# Autodesk Inventor assembly: SPE1V1 Estructura
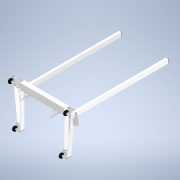
[picture p0: Inventor's stored thumbnail of the model, 180x180]
Saved by Autodesk Inventor 2021.2 (Build 252289000, 289)
## iProperties
Created: 2026-06-02
Part Number: SPE1V1 Estructura
Document SubType Name: Assembly
Designer: nelso
Author: nelso
## Documents named in this file (15)
- C:\Users\nelso\Desktop\Soporte-Paciente-Espinografia\Workspace\SPE1V1 Estructura.iam
- C:\Users\nelso\Desktop\Soporte-Paciente-Espinografia\Workspace\SP22V1 Tubo 40x80x1825mm.ipt
- C:\Users\nelso\Desktop\Soporte-Paciente-Espinografia\Workspace\SP21V1 Tubo 40x80x100mm.ipt
- C:\Users\nelso\Desktop\Soporte-Paciente-Espinografia\Workspace\SPE4V1 Rueda.iam
- C:\Users\nelso\Desktop\Soporte-Paciente-Espinografia\Workspace\SP23V1 Cobertora Derecha.ipt
- C:\Users\nelso\Desktop\Soporte-Paciente-Espinografia\Workspace\SP24V1 Cobertora Izquierda.ipt
- C:\Users\nelso\Desktop\Soporte-Paciente-Espinografia\Workspace\SP20V1 Tubo 80x120x790mm.ipt
- C:\Users\nelso\Desktop\Soporte-Paciente-Espinografia\Workspace\SP19V1 Tapacanto Delantero.ipt
- C:\Users\nelso\Desktop\Soporte-Paciente-Espinografia\Workspace\SP18V1 Tapacanto Superior.ipt
- C:\Users\nelso\Desktop\Soporte-Paciente-Espinografia\Workspace\RFPLUS8PO300.ipt
- C:\Users\nelso\Desktop\Soporte-Paciente-Espinografia\Workspace\SP17V1 Varilla Pedal.ipt
- C:\Users\nelso\Desktop\Soporte-Paciente-Espinografia\Workspace\SP16V1 Buje Pedal.ipt
- C:\Users\nelso\Desktop\Soporte-Paciente-Espinografia\Workspace\SP15V1 Pedal Izquierdo.ipt
- C:\Users\nelso\Desktop\Soporte-Paciente-Espinografia\Workspace\SPE3V1 Freno.iam
- C:\Users\nelso\Desktop\Soporte-Paciente-Espinografia\Workspace\SP14V1 Pedal Derecho.ipt
## Components (40 placed, 14 different names)
1. tubo2-40x40x1800:1 — Nivelación:17, Coincidencia:54, Coincidencia:55, Coincidencia:68, Nivelación:67, Coincidencia:71, Flush:75, Flush:76, Flush:77, Flush:78, Flush:79, Mate:84, Mate:85, Mate:86, Mate:87, Mate:88, Mate:107, Flush:101
2. tubo2-40x40x1800:2 — Flush:115, Mate:143, Mate:144
3. SPE21V1 Tubo 40x80x100mm:1 — Mate:15, Nivelación:14, Coincidencia:24, Coincidencia:30, Coincidencia:42, Coincidencia:60, Coincidencia:62, Coincidencia:63
4. SPE21V1 Tubo 40x80x100mm:2 — Coincidencia:37, Coincidencia:38, Coincidencia:40, Coincidencia:41, Coincidencia:66
5. SPE21V1 Tubo 40x80x100mm:3 — Coincidencia:48, Coincidencia:49, Coincidencia:50, Coincidencia:51, Coincidencia:65
6. SPE21V1 Tubo 40x80x100mm:4 — Mate:150, Mate:151
7. SPE4V1 Rueda:1 [sub-assembly] — Coincidencia:48, Coincidencia:49
8. SPE4V1 Rueda:3 [sub-assembly] — Coincidencia:40, Coincidencia:41
9. SPE4V1 Rueda:4 [sub-assembly] — Mate:15, Coincidencia:30
10. SPE4V1 Rueda:5 [sub-assembly]
11. SP23V1 Cobertora Derecha:1 — Nivelación:14, Coincidencia:24, Nivelación:17, Coincidencia:37, Coincidencia:38, Nivelación:18, Coincidencia:42, Nivelación:26, Coincidencia:55, Nivelación:27, Coincidencia:66, Flush:97, Flush:98, Mate:96, Mate:97, Flush:105, Mate:126, Mate:131
12. SP22V1 Cobertora Izquierda:1 — Nivelación:18, Coincidencia:50, Coincidencia:51, Nivelación:24, Coincidencia:53, Nivelación:28, Coincidencia:65, Flush:95, Flush:96, Mate:94, Mate:95, Flush:104, Mate:127, Flush:115, Mate:143, Mate:144, Mate:150, Mate:151, Mate:152
13. tubo3-40x80x800:1 — Nivelación:24, Nivelación:25, Coincidencia:54, Nivelación:27, Nivelación:28, Mate:110, Mate:111, Mate:124
14. SP19V1 Tapacanto Delantero:1 — Coincidencia:60, Coincidencia:62, Coincidencia:63
15. SP18V1 Tapacanto Superior:1 — Coincidencia:68, Nivelación:67, Coincidencia:71
16. RFPLUS8PO300:1 — Mate:107, Flush:101
17. RFPLUS8PO300:2 — Flush:75, Mate:88
18. RFPLUS8PO300:3 — Flush:76, Mate:87
19. RFPLUS8PO300:4 — Flush:77, Mate:86
20. RFPLUS8PO300:5 — Flush:78, Mate:84
21. RFPLUS8PO300:6 — Flush:79, Mate:85
22. RFPLUS8PO300:13 — Flush:95, Mate:94
23. RFPLUS8PO300:14 — Flush:96, Mate:95
24. RFPLUS8PO300:15 — Flush:97, Mate:97
25. RFPLUS8PO300:16 — Flush:98, Mate:96
26. SP17V1 Varilla Pedal:1 — Flush:102, Mate:117, Mate:118, Mate:119, Mate:120, Mate:121, Mate:125, Mate:128, Mate:129, Mate:130, Mate:132, Mate:133, Mate:134, Flush:106, Flush:107
27. SP16V1 Buje Pedal:1 — Mate:116, Flush:105, Mate:131
28. SP16V1 Buje Pedal:2 — Mate:116, Mate:125, Flush:104
29. SP15V1 Pedal Izquierdo:1 — Mate:120, Mate:121, Flush:106
30. SPE3V1 Freno:1 [sub-assembly] — Mate:110, Flush:103, Mate:117, Mate:118, Mate:119, Mate:124, Mate:127
31. SPE3V1 Freno:2 [sub-assembly] — Mate:111, Flush:103, Mate:126, Mate:133, Mate:134
32. SP14V1 Pedal Derecho:1 — Mate:128, Mate:129, Mate:130, Mate:132, Flush:107
33. SP18V1 Tapacanto Superior:2
34. RFPLUS8PO300:17
35. RFPLUS8PO300:18
36. RFPLUS8PO300:19
37. RFPLUS8PO300:20
38. RFPLUS8PO300:21
39. RFPLUS8PO300:22
40. SP19V1 Tapacanto Delantero:2 — Mate:152
## Relationships (102: Mate 69, Flush 33)
- Mate:15: SPE21V1 Tubo 40x80x100mm:1 ↔ SPE4V1 Rueda:4
- Nivelación:14 [Flush]: SPE21V1 Tubo 40x80x100mm:1 ↔ SP23V1 Cobertora Derecha:1
- Coincidencia:24 [Mate] (0.5 mm): SPE21V1 Tubo 40x80x100mm:1 ↔ SP23V1 Cobertora Derecha:1
- Coincidencia:30 [Mate]: SPE21V1 Tubo 40x80x100mm:1 ↔ SPE4V1 Rueda:4
- Nivelación:17 [Flush]: tubo2-40x40x1800:1 ↔ SP23V1 Cobertora Derecha:1
- Coincidencia:37 [Mate]: SPE21V1 Tubo 40x80x100mm:2 ↔ SP23V1 Cobertora Derecha:1
- Coincidencia:38 [Mate]: SPE21V1 Tubo 40x80x100mm:2 ↔ SP23V1 Cobertora Derecha:1
- Coincidencia:40 [Mate]: SPE21V1 Tubo 40x80x100mm:2 ↔ SPE4V1 Rueda:3
- Coincidencia:41 [Mate]: SPE21V1 Tubo 40x80x100mm:2 ↔ SPE4V1 Rueda:3
- Nivelación:18 [Flush]: SP23V1 Cobertora Derecha:1 ↔ SP22V1 Cobertora Izquierda:1
- Coincidencia:42 [Mate]: SPE21V1 Tubo 40x80x100mm:1 ↔ SP23V1 Cobertora Derecha:1
- Coincidencia:48 [Mate]: SPE21V1 Tubo 40x80x100mm:3 ↔ SPE4V1 Rueda:1
- Coincidencia:49 [Mate]: SPE21V1 Tubo 40x80x100mm:3 ↔ SPE4V1 Rueda:1
- Coincidencia:50 [Mate]: SPE21V1 Tubo 40x80x100mm:3 ↔ SP22V1 Cobertora Izquierda:1
- Coincidencia:51 [Mate]: SPE21V1 Tubo 40x80x100mm:3 ↔ SP22V1 Cobertora Izquierda:1
- Nivelación:24 [Flush]: SP22V1 Cobertora Izquierda:1 ↔ tubo3-40x80x800:1
- Nivelación:25 [Flush]: tubo3-40x80x800:1
- Coincidencia:53 [Mate] (395 mm): SP22V1 Cobertora Izquierda:1
- Nivelación:26 [Flush] (395 mm): SP23V1 Cobertora Derecha:1
- Coincidencia:54 [Mate]: tubo2-40x40x1800:1 ↔ tubo3-40x80x800:1
- Coincidencia:55 [Mate]: tubo2-40x40x1800:1 ↔ SP23V1 Cobertora Derecha:1
- Nivelación:27 [Flush]: SP23V1 Cobertora Derecha:1 ↔ tubo3-40x80x800:1
- Nivelación:28 [Flush]: SP22V1 Cobertora Izquierda:1 ↔ tubo3-40x80x800:1
- Coincidencia:60 [Mate]: SPE21V1 Tubo 40x80x100mm:1 ↔ SP19V1 Tapacanto Delantero:1
- Coincidencia:62 [Mate]: SPE21V1 Tubo 40x80x100mm:1 ↔ SP19V1 Tapacanto Delantero:1
- Coincidencia:63 [Mate]: SPE21V1 Tubo 40x80x100mm:1 ↔ SP19V1 Tapacanto Delantero:1
- Coincidencia:65 [Mate]: SPE21V1 Tubo 40x80x100mm:3 ↔ SP22V1 Cobertora Izquierda:1
- Coincidencia:66 [Mate]: SPE21V1 Tubo 40x80x100mm:2 ↔ SP23V1 Cobertora Derecha:1
- Coincidencia:68 [Mate]: tubo2-40x40x1800:1 ↔ SP18V1 Tapacanto Superior:1
- Nivelación:67 [Flush]: tubo2-40x40x1800:1 ↔ SP18V1 Tapacanto Superior:1
- Coincidencia:71 [Mate]: tubo2-40x40x1800:1 ↔ SP18V1 Tapacanto Superior:1
- Flush:75: tubo2-40x40x1800:1 ↔ RFPLUS8PO300:2
- Flush:76: tubo2-40x40x1800:1 ↔ RFPLUS8PO300:3
- Flush:77: tubo2-40x40x1800:1 ↔ RFPLUS8PO300:4
- Flush:78: tubo2-40x40x1800:1 ↔ RFPLUS8PO300:5
- Flush:79: tubo2-40x40x1800:1 ↔ RFPLUS8PO300:6
- Mate:84: tubo2-40x40x1800:1 ↔ RFPLUS8PO300:5
- Mate:85: tubo2-40x40x1800:1 ↔ RFPLUS8PO300:6
- Mate:86: tubo2-40x40x1800:1 ↔ RFPLUS8PO300:4
- Mate:87: tubo2-40x40x1800:1 ↔ RFPLUS8PO300:3
- Mate:88: tubo2-40x40x1800:1 ↔ RFPLUS8PO300:2
- Flush:95: SP22V1 Cobertora Izquierda:1 ↔ RFPLUS8PO300:13
- Flush:96: SP22V1 Cobertora Izquierda:1 ↔ RFPLUS8PO300:14
- Mate:94: SP22V1 Cobertora Izquierda:1 ↔ RFPLUS8PO300:13
- Mate:95: SP22V1 Cobertora Izquierda:1 ↔ RFPLUS8PO300:14
- Flush:97: SP23V1 Cobertora Derecha:1 ↔ RFPLUS8PO300:15
- Flush:98: SP23V1 Cobertora Derecha:1 ↔ RFPLUS8PO300:16
- Mate:96: SP23V1 Cobertora Derecha:1 ↔ RFPLUS8PO300:16
- Mate:97: SP23V1 Cobertora Derecha:1 ↔ RFPLUS8PO300:15
- Mate:107: tubo2-40x40x1800:1 ↔ RFPLUS8PO300:1
- Flush:101: tubo2-40x40x1800:1 ↔ RFPLUS8PO300:1
- Flush:102: SP17V1 Varilla Pedal:1
- Mate:110: tubo3-40x80x800:1 ↔ SPE3V1 Freno:1
- Mate:111: tubo3-40x80x800:1 ↔ SPE3V1 Freno:2
- Mate:116: SP16V1 Buje Pedal:1 ↔ SP16V1 Buje Pedal:2
- Flush:103: SPE3V1 Freno:1 ↔ SPE3V1 Freno:2
- Mate:117: SP17V1 Varilla Pedal:1 ↔ SPE3V1 Freno:1
- Mate:118: SP17V1 Varilla Pedal:1 ↔ SPE3V1 Freno:1
- Mate:119: SP17V1 Varilla Pedal:1 ↔ SPE3V1 Freno:1
- Mate:120: SP17V1 Varilla Pedal:1 ↔ SP15V1 Pedal Izquierdo:1
- Mate:121: SP17V1 Varilla Pedal:1 ↔ SP15V1 Pedal Izquierdo:1
- Mate:124: tubo3-40x80x800:1 ↔ SPE3V1 Freno:1
- Mate:125: SP17V1 Varilla Pedal:1 ↔ SP16V1 Buje Pedal:2
- Flush:104: SP22V1 Cobertora Izquierda:1 ↔ SP16V1 Buje Pedal:2
- Flush:105: SP23V1 Cobertora Derecha:1 ↔ SP16V1 Buje Pedal:1
- Mate:126 (100 mm): SP23V1 Cobertora Derecha:1 ↔ SPE3V1 Freno:2
- Mate:127 (100 mm): SP22V1 Cobertora Izquierda:1 ↔ SPE3V1 Freno:1
- Mate:128: SP17V1 Varilla Pedal:1 ↔ SP14V1 Pedal Derecho:1
- Mate:129: SP17V1 Varilla Pedal:1 ↔ SP14V1 Pedal Derecho:1
- Mate:130: SP17V1 Varilla Pedal:1 ↔ SP14V1 Pedal Derecho:1
- Mate:131: SP23V1 Cobertora Derecha:1 ↔ SP16V1 Buje Pedal:1
- Mate:132: SP17V1 Varilla Pedal:1 ↔ SP14V1 Pedal Derecho:1
- Mate:133: SP17V1 Varilla Pedal:1 ↔ SPE3V1 Freno:2
- Mate:134: SP17V1 Varilla Pedal:1 ↔ SPE3V1 Freno:2
- Flush:106: SP17V1 Varilla Pedal:1 ↔ SP15V1 Pedal Izquierdo:1
- Flush:107: SP17V1 Varilla Pedal:1 ↔ SP14V1 Pedal Derecho:1
- [Mate]: tubo2-40x40x1800:2 ↔ SP18V1 Tapacanto Superior:2
- [Flush]: tubo2-40x40x1800:2 ↔ SP18V1 Tapacanto Superior:2
- [Mate]: tubo2-40x40x1800:2 ↔ SP18V1 Tapacanto Superior:2
- [Flush]: tubo2-40x40x1800:2 ↔ RFPLUS8PO300:18
- [Flush]: tubo2-40x40x1800:2 ↔ RFPLUS8PO300:19
- [Flush]: tubo2-40x40x1800:2 ↔ RFPLUS8PO300:20
- [Flush]: tubo2-40x40x1800:2 ↔ RFPLUS8PO300:21
- [Flush]: tubo2-40x40x1800:2 ↔ RFPLUS8PO300:22
- [Mate]: tubo2-40x40x1800:2 ↔ RFPLUS8PO300:21
- [Mate]: tubo2-40x40x1800:2 ↔ RFPLUS8PO300:22
- [Mate]: tubo2-40x40x1800:2 ↔ RFPLUS8PO300:20
- [Mate]: tubo2-40x40x1800:2 ↔ RFPLUS8PO300:19
- [Mate]: tubo2-40x40x1800:2 ↔ RFPLUS8PO300:18
- [Mate]: tubo2-40x40x1800:2 ↔ RFPLUS8PO300:17
- [Flush]: tubo2-40x40x1800:2 ↔ RFPLUS8PO300:17
- Flush:115: tubo2-40x40x1800:2 ↔ SP22V1 Cobertora Izquierda:1
- Mate:143: tubo2-40x40x1800:2 ↔ SP22V1 Cobertora Izquierda:1
- Mate:144: tubo2-40x40x1800:2 ↔ SP22V1 Cobertora Izquierda:1
- [Mate]: SPE21V1 Tubo 40x80x100mm:4 ↔ SPE4V1 Rueda:5
- [Mate]: SPE21V1 Tubo 40x80x100mm:4 ↔ SPE4V1 Rueda:5
- [Mate]: SPE21V1 Tubo 40x80x100mm:4 ↔ SP19V1 Tapacanto Delantero:2
- [Mate]: SPE21V1 Tubo 40x80x100mm:4 ↔ SP19V1 Tapacanto Delantero:2
- [Mate]: SPE21V1 Tubo 40x80x100mm:4 ↔ SP19V1 Tapacanto Delantero:2
- Mate:150 (0.5 mm): SPE21V1 Tubo 40x80x100mm:4 ↔ SP22V1 Cobertora Izquierda:1
- Mate:151: SPE21V1 Tubo 40x80x100mm:4 ↔ SP22V1 Cobertora Izquierda:1
- Mate:152: SP22V1 Cobertora Izquierda:1 ↔ SP19V1 Tapacanto Delantero:2
## Named parameters: d303_d128 = 0 mm, d304_d129 = 0 mm, d305_d130 = 0 mm, d306_d131 = 0 mm, d307_d132 = 0 mm, d308_d133 = 0 mm, d309_d134 = 0 mm, d310_d135 = 0 mm, d311_d213 = 0 mm, d312_d214 = 0 mm, d313_d99 = 0 mm, d314_d103 = 0 mm, d315_d104 = 0 mm, d316_d126 = 0 mm, d317_d127 = 0 mm, d329_d21 = 0 mm, d330_d90 = 0 mm, d331_d92 = 0 mm, d332_d93 = 0 mm, d333_d43 = 0 mm
